# Autodesk Inventor assembly: 18650_assembly
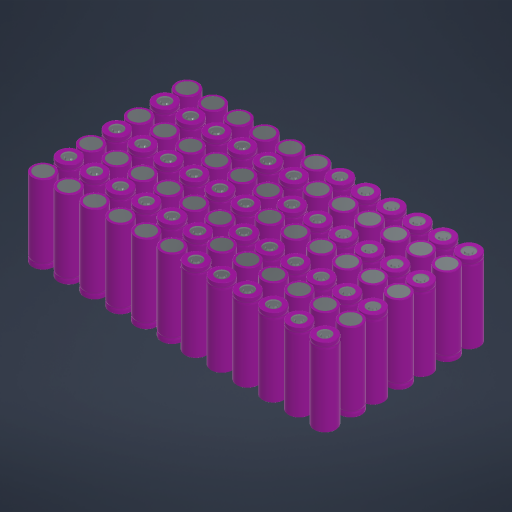
[picture p0: Inventor's stored thumbnail of the model, 512x512]
Saved by Autodesk Inventor 2024.3 (Build 283343010, 343A)
## iProperties
Created: 2025-05-07
Part Number: 18650_assembly
Document SubType Name: Assembly
Designer: David
Author: David
## Documents named in this file (2)
- C:\Users\David\Documents\FTAG\E-16\Batterie\Batterie_Konstruktion\E-16 Batterie\18650_assembly.iam
- C:\Users\David\Documents\FTAG\E-16\Batterie\Batterie_Konstruktion\E-16 Batterie\18650.ipt
## Components (84 placed, 1 different names)
1. 18650:19 — Tangential:1, Tangential:3, Passend:1, Fluchtend:1
2. 18650:20
3. 18650:21
4. 18650:22
5. 18650:23
6. 18650:24
7. 18650:25
8. 18650:26
9. 18650:27
10. 18650:28
11. 18650:29
12. 18650:30
13. 18650:31
14. 18650:32
15. 18650:33
16. 18650:34
17. 18650:35
18. 18650:36
19. 18650:37
20. 18650:38
21. 18650:39
22. 18650:40
23. 18650:41
24. 18650:42
25. 18650:1 — Tangential:2, Tangential:4, Fluchtend:1
26. 18650:2
27. 18650:3
28. 18650:4
29. 18650:5
30. 18650:6
31. 18650:7
32. 18650:8
33. 18650:9
34. 18650:10
35. 18650:11
36. 18650:12
37. 18650:13
38. 18650:14
39. 18650:15
40. 18650:16
41. 18650:17
42. 18650:18
43. 18650:43
44. 18650:44
45. 18650:45
46. 18650:46
47. 18650:47
48. 18650:48
49. 18650:49
50. 18650:50
51. 18650:51
52. 18650:52
53. 18650:53
54. 18650:54
55. 18650:55
56. 18650:56
57. 18650:57
58. 18650:58
59. 18650:59
60. 18650:60
61. 18650:61
62. 18650:62
63. 18650:63
64. 18650:64
65. 18650:65
66. 18650:66
67. 18650:67
68. 18650:68
69. 18650:69
70. 18650:70
71. 18650:71
72. 18650:72
73. 18650:73
74. 18650:74
75. 18650:75
76. 18650:76
77. 18650:77
78. 18650:78
79. 18650:79
80. 18650:80
81. 18650:81
82. 18650:82
83. 18650:83
84. 18650:84
## Component patterns: (2 elements), (24 elements, first: 18650:19), (18 elements, first: 18650:1), Komponentenanordnung 2:2 (24 elements), Komponentenanordnung 1:2 (18 elements)
## Relationships (6: Tangent 4, Mate 1, Flush 1)
- Tangential:1 (1 mm): 18650:19
- Tangential:2 (1 mm): 18650:1
- Tangential:3: 18650:19
- Tangential:4 (21.5 mm): 18650:1
- Passend:1 [Mate] (-32.5 mm): 18650:19
- Fluchtend:1 [Flush]: 18650:19 ↔ 18650:1
